# Autodesk Inventor assembly: Fahrgestell_Baugruppe_01
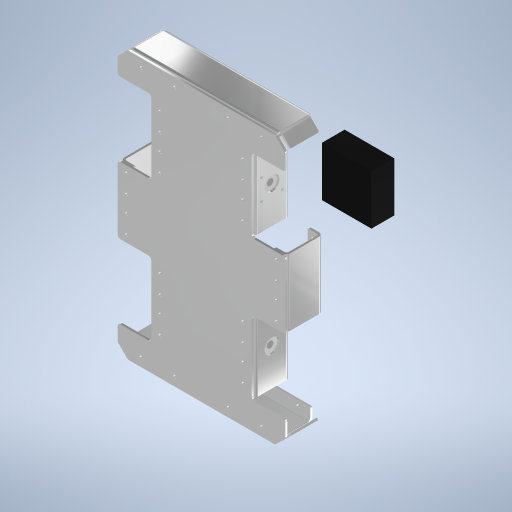
[picture p0: Inventor's stored thumbnail of the model, 512x512]
Saved by Autodesk Inventor 2024 (Build 280153000, 153)
## iProperties
Created: 2024-03-25
Part Number: Fahrgestell_Baugruppe_01
Document SubType Name: Assembly
Designer: month
Mass: 1363.96 g
Surface Area: 3580.03 cm^2
Volume: 505.169 cm^3
Density: 2.7 g/cm^3
Author: month
## Documents named in this file (8)
- C:\Users\month\Documents\Inventor\Elektronische_Produktentwicklung_FF-Tank\Fahrgestell_Baugruppe_01.iam
- C:\Users\month\Documents\Inventor\Elektronische_Produktentwicklung_FF-Tank\Grundgehäuse_01.ipt
- C:\Users\month\Documents\Inventor\Elektronische_Produktentwicklung_FF-Tank\Motorhalter_02.ipt
- C:\Users\month\Documents\Inventor\Elektronische_Produktentwicklung_FF-Tank\Seitenteil_03.ipt
- C:\Users\month\Documents\Inventor\Elektronische_Produktentwicklung_FF-Tank\Stossfänger_04.ipt
- C:\Users\month\Documents\Inventor\Elektronische_Produktentwicklung_FF-Tank\Motor.ipt
- C:\Users\month\Documents\Inventor\Elektronische_Produktentwicklung_FF-Tank\Platine.ipt
- C:\Users\month\Documents\Inventor\Elektronische_Produktentwicklung_FF-Tank\DCDC_Wandler.ipt
## Components (16 placed, 7 different names)
1. Grundgehäuse_01:1 — Passend:2, Passend:3, Passend:5, Passend:6, Passend:8, Passend:9, Passend:11, Passend:12, Passend:13, Passend:14, Passend:15, Passend:16, Passend:17, Passend:18, Passend:19, Passend:20, Passend:21, Passend:22, Passend:23, Passend:24, Passend:25, Passend:26, Passend:27, Passend:28, Passend:37
2. Motorhalter_02:1 — Passend:2, Passend:3, Passend:13, Passend:34, Einfügen:1
3. Motorhalter_02:2 — Passend:5, Passend:6, Passend:14, Passend:35, Einfügen:3
4. Motorhalter_02:3 — Passend:8, Passend:9, Passend:16, Passend:36, Einfügen:2
5. Motorhalter_02:4 — Passend:11, Passend:12, Passend:15, Passend:32, Passend:33
6. Seitenteil_03:1 — Passend:17, Passend:18, Passend:19, Fluchtend:1
7. Seitenteil_03:2 — Passend:20, Passend:21, Passend:22
8. Stossfänger_04:1 — Passend:23, Passend:24, Passend:25, Passend:29, Passend:30
9. Stossfänger_04:2 — Passend:26, Passend:27, Passend:28, Passend:31
10. Grundgehäuse_01:2 — Passend:29, Passend:30, Passend:31
11. Motor:1 — Passend:32, Passend:33
12. Motor:2 — Passend:35, Einfügen:3
13. Motor:3 — Passend:34, Einfügen:1
14. Motor:4 — Passend:36, Einfügen:2
15. Platine:1 — Passend:37
16. DCDC_Wandler:1 — Fluchtend:1
## Relationships (37: Mate 33, Insert 3, Flush 1)
- Passend:2 [Mate]: Grundgehäuse_01:1 ↔ Motorhalter_02:1
- Passend:3 [Mate]: Grundgehäuse_01:1 ↔ Motorhalter_02:1
- Passend:5 [Mate]: Grundgehäuse_01:1 ↔ Motorhalter_02:2
- Passend:6 [Mate]: Grundgehäuse_01:1 ↔ Motorhalter_02:2
- Passend:8 [Mate]: Grundgehäuse_01:1 ↔ Motorhalter_02:3
- Passend:9 [Mate]: Grundgehäuse_01:1 ↔ Motorhalter_02:3
- Passend:11 [Mate]: Grundgehäuse_01:1 ↔ Motorhalter_02:4
- Passend:12 [Mate]: Grundgehäuse_01:1 ↔ Motorhalter_02:4
- Passend:13 [Mate]: Grundgehäuse_01:1 ↔ Motorhalter_02:1
- Passend:14 [Mate]: Grundgehäuse_01:1 ↔ Motorhalter_02:2
- Passend:15 [Mate]: Grundgehäuse_01:1 ↔ Motorhalter_02:4
- Passend:16 [Mate]: Grundgehäuse_01:1 ↔ Motorhalter_02:3
- Passend:17 [Mate]: Grundgehäuse_01:1 ↔ Seitenteil_03:1
- Passend:18 [Mate]: Grundgehäuse_01:1 ↔ Seitenteil_03:1
- Passend:19 [Mate]: Grundgehäuse_01:1 ↔ Seitenteil_03:1
- Passend:20 [Mate]: Grundgehäuse_01:1 ↔ Seitenteil_03:2
- Passend:21 [Mate]: Grundgehäuse_01:1 ↔ Seitenteil_03:2
- Passend:22 [Mate]: Grundgehäuse_01:1 ↔ Seitenteil_03:2
- Passend:23 [Mate]: Grundgehäuse_01:1 ↔ Stossfänger_04:1
- Passend:24 [Mate]: Grundgehäuse_01:1 ↔ Stossfänger_04:1
- Passend:25 [Mate]: Grundgehäuse_01:1 ↔ Stossfänger_04:1
- Passend:26 [Mate]: Grundgehäuse_01:1 ↔ Stossfänger_04:2
- Passend:27 [Mate]: Grundgehäuse_01:1 ↔ Stossfänger_04:2
- Passend:28 [Mate]: Grundgehäuse_01:1 ↔ Stossfänger_04:2
- Passend:29 [Mate]: Stossfänger_04:1 ↔ Grundgehäuse_01:2
- Passend:30 [Mate]: Stossfänger_04:1 ↔ Grundgehäuse_01:2
- Passend:31 [Mate]: Stossfänger_04:2 ↔ Grundgehäuse_01:2
- Passend:32 [Mate]: Motorhalter_02:4 ↔ Motor:1
- Passend:33 [Mate]: Motorhalter_02:4 ↔ Motor:1
- Passend:34 [Mate]: Motorhalter_02:1 ↔ Motor:3
- Passend:35 [Mate]: Motorhalter_02:2 ↔ Motor:2
- Passend:36 [Mate]: Motorhalter_02:3 ↔ Motor:4
- Einfügen:1 [Insert]: Motorhalter_02:1 ↔ Motor:3
- Einfügen:2 [Insert]: Motorhalter_02:3 ↔ Motor:4
- Einfügen:3 [Insert]: Motorhalter_02:2 ↔ Motor:2
- Passend:37 [Mate]: Grundgehäuse_01:1 ↔ Platine:1
- Fluchtend:1 [Flush]: Seitenteil_03:1 ↔ DCDC_Wandler:1
